# Autodesk Inventor assembly: base_bearingpole_front_MIR_assy
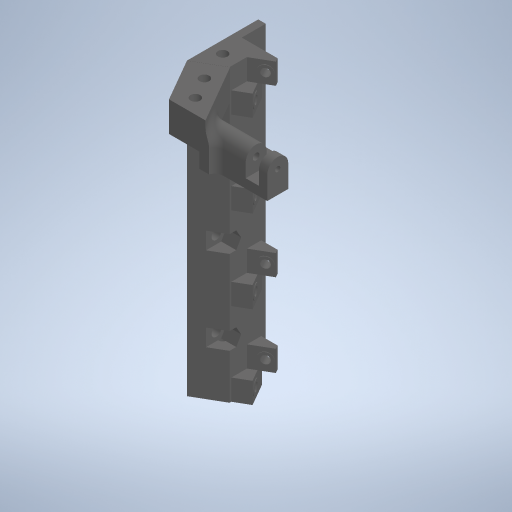
[picture p0: Inventor's stored thumbnail of the model, 512x512]
Saved by Autodesk Inventor 2024.1 (Build 281209000, 209)
## iProperties
Created: 2025-03-04
Part Number: base_bearingpole_front_MIR_assy
Document SubType Name: Assembly
Designer: hibik
Author: hibik
## Documents named in this file (3)
- C:\Users\hibik\Documents\Robomech\RESCUE\ORCA\hard\fork\right\base_bearingpole_front_MIR_assy.iam
- C:\Users\hibik\Documents\Robomech\RESCUE\ORCA\hard\fork\right\base_bearingpole_front_MIR.ipt
- C:\Users\hibik\Documents\Robomech\RESCUE\ORCA\hard\fork\right\chain_base_connector_MIR.ipt
## Components (2 placed, 2 different names)
1. base_bearingpole_front_MIR:1 — メイト:1, フラッシュ:1, メイト:2
2. chain_base_connector_MIR:1 — メイト:1, フラッシュ:1, メイト:2
## Relationships (3: Mate 2, Flush 1)
- メイト:1 [Mate]: base_bearingpole_front_MIR:1 ↔ chain_base_connector_MIR:1
- フラッシュ:1 [Flush]: base_bearingpole_front_MIR:1 ↔ chain_base_connector_MIR:1
- メイト:2 [Mate]: base_bearingpole_front_MIR:1 ↔ chain_base_connector_MIR:1
